# Autodesk Inventor assembly: INTERFACE 2
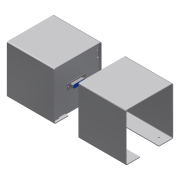
[picture p0: Inventor's stored thumbnail of the model, 180x180]
Saved by Autodesk Inventor 2018 (Build 220112000, 112)
## iProperties
Created: 2018-12-19
Part Number: INTERFACE 2
Document SubType Name: Assembly
Designer: R.P.SMITH
Mass: 378.434 g
Surface Area: 1950.63 cm^2
Volume: 143.625 cm^3
Density: 2.63487 g/cm^3
Author: R.P.SMITH
## Documents named in this file (5)
- D:\Documents\College\Semesters\4 - Fall\Senior Project 2\CADD Files\INTERFACE 2.iam
- D:\Documents\College\Semesters\4 - Fall\Senior Project 2\CADD Files\Custom Parts\SEGMENT SHELL.ipt
- D:\Documents\College\Semesters\4 - Fall\Senior Project 2\CADD Files\Custom Parts\END MOUNT INTERFACE 2.iam
- D:\Documents\College\Semesters\4 - Fall\Senior Project 2\CADD Files\Custom Parts\D SUB 15P female Threaded - FLT15S7-K121 (FCT).ipt
- D:\Documents\College\Semesters\4 - Fall\Senior Project 2\CADD Files\Custom Parts\D SUB 15P male Threaded - FLT15P7-K120 (FCT).ipt
## Components (6 placed, 4 different names)
1. SEGMENT SHELL:1 — Mate:1, Mate:2, Flush:1, Flush:2, Flush:3
2. END MOUNT INTERFACE 2:1 [sub-assembly] — Mate:1, Mate:2, Mate:3, Mate:4, Mate:5, Flush:1
3. D SUB 15P female Threaded - FLT15S7-K121 (FCT):1 — Mate:3, Mate:4, Mate:5
4. D SUB 15P male Threaded - FLT15P7-K120 (FCT):1 — Mate:8, Mate:9, Mate:10
5. SEGMENT SHELL:2 — Flush:2, Flush:3, Mate:6, Mate:7, Flush:4
6. END MOUNT INTERFACE 2:2 [sub-assembly] — Mate:6, Mate:7, Mate:8, Mate:9, Mate:10, Flush:4
## Relationships (14: Mate 10, Flush 4)
- Mate:1 (0.25 mm): SEGMENT SHELL:1 ↔ END MOUNT INTERFACE 2:1
- Mate:2 (0.25 mm): SEGMENT SHELL:1 ↔ END MOUNT INTERFACE 2:1
- Mate:3: END MOUNT INTERFACE 2:1 ↔ D SUB 15P female Threaded - FLT15S7-K121 (FCT):1
- Mate:4: END MOUNT INTERFACE 2:1 ↔ D SUB 15P female Threaded - FLT15S7-K121 (FCT):1
- Mate:5: END MOUNT INTERFACE 2:1 ↔ D SUB 15P female Threaded - FLT15S7-K121 (FCT):1
- Flush:1 (4 mm): SEGMENT SHELL:1 ↔ END MOUNT INTERFACE 2:1
- Flush:2: SEGMENT SHELL:1 ↔ SEGMENT SHELL:2
- Flush:3: SEGMENT SHELL:1 ↔ SEGMENT SHELL:2
- Mate:6 (0.25 mm): SEGMENT SHELL:2 ↔ END MOUNT INTERFACE 2:2
- Mate:7 (0.25 mm): SEGMENT SHELL:2 ↔ END MOUNT INTERFACE 2:2
- Mate:8: D SUB 15P male Threaded - FLT15P7-K120 (FCT):1 ↔ END MOUNT INTERFACE 2:2
- Mate:9: D SUB 15P male Threaded - FLT15P7-K120 (FCT):1 ↔ END MOUNT INTERFACE 2:2
- Mate:10: D SUB 15P male Threaded - FLT15P7-K120 (FCT):1 ↔ END MOUNT INTERFACE 2:2
- Flush:4 (4 mm): SEGMENT SHELL:2 ↔ END MOUNT INTERFACE 2:2
